# Autodesk Inventor assembly: Guidler Assembly
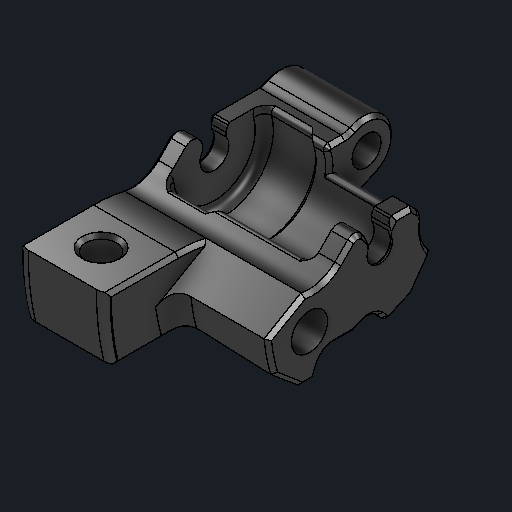
[picture p0: Inventor's stored thumbnail of the model, 512x512]
Saved by Autodesk Inventor 2026.1 (Build 301233020, 233B)
## iProperties
Created: 2025-05-11
Part Number: Guidler Assembly
Document SubType Name: Assembly
Designer: Joshua Eah
Author: Joshua Eah
## Documents named in this file (3)
- C:\Users\JoshuaEah\Documents\GitHub\Voron-0\CAD\Toolhead\Subassemblies\Guidler Assembly.iam
- C:\Users\JoshuaEah\Documents\GitHub\Voron-0\CAD\Hardware\M2x10 Self Tapper.ipt
- C:\Users\JoshuaEah\Documents\GitHub\Voron-0\CAD\Toolhead\Parts\Toolhead Frame\Guidler.ipt
## Components (2 placed, 2 different names)
1. M2x10 Self Tapper:1
2. Guidler:1
## Relationships (1: Insert 1)
- [Insert]: M2x10 Self Tapper:1 ↔ Guidler:1
